# Autodesk Inventor assembly: Assembly1
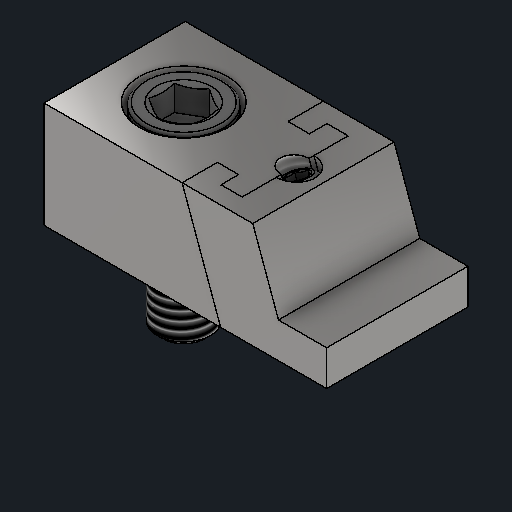
[picture p0: Inventor's stored thumbnail of the model, 512x512]
Saved by Autodesk Inventor 2026.2 (Build 302298000, 298)
## iProperties
Created: 2026-09-23
Part Number: Assembly1
Document SubType Name: Assembly
Designer: JoshuaEah
Author: JoshuaEah
## Documents named in this file (5)
- C:\Users\Joshua Eah\Documents\GitHub\designs\Toe Clamps\Low Profile Side Clamp.iam
- C:\Users\Joshua Eah\Documents\GitHub\designs\Toe Clamps\Fixed Base.ipt
- C:\Users\Joshua Eah\Documents\GitHub\designs\Toe Clamps\Moving Jaw (Clearance Cut).ipt
- C:\Users\Joshua Eah\Documents\GitHub\designs\Toe Clamps\0.25-20x0.5 Set Screw.ipt
- C:\Users\Joshua Eah\Documents\GitHub\designs\Toe Clamps\3-8-16x1 SHCS.ipt
## Components (4 placed, 4 different names)
1. Fixed Base:1 — Mate:1, Insert:2, Slider:1
2. Moving Jaw (Clearance Cut):1 — Insert:3, Slider:1
3. 0.25-20x0.5 Set Screw:1 — Mate:1, Insert:3
4. 3-8-16x1 SHCS:1 — Insert:2
## Relationships (4: Insert 2, Mate 1, TranslationJoint 1)
- Mate:1: Fixed Base:1 ↔ 0.25-20x0.5 Set Screw:1
- Insert:2: Fixed Base:1 ↔ 3-8-16x1 SHCS:1
- Insert:3: Moving Jaw (Clearance Cut):1 ↔ 0.25-20x0.5 Set Screw:1
- Slider:1 [TranslationJoint]: Fixed Base:1 ↔ Moving Jaw (Clearance Cut):1
